# Autodesk Inventor assembly: Eto_Project
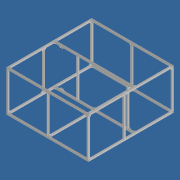
[picture p0: Inventor's stored thumbnail of the model, 180x180]
Saved by Autodesk Inventor 2020 (Build 240168000, 168)
## iProperties
Created: 2021-06-15
Part Number: Eto_Project
Description: CAx-IF Rec.Pracs.---Model Styling and Organization---1.2---2011-12-15
Document SubType Name: Assembly
Designer: ken113
Sending System: 3D_Kernel_IO2017 Sp2 by CT CoreTechnologie
Preprocessor: STEP Interface 2017 Sp2 by CT CoreTechnologie
Title: Eto_Project.stp
## Documents named in this file (68)
- D:\Document\Github\Eto_Project\Hardware\Asem\FRAMES\FramesEto_Project.iam
- D:\Document\Github\Eto_Project\Hardware\Asem\FRAMES\FramesHFS6-3030-1500.ipt
- D:\Document\Github\Eto_Project\Hardware\Asem\FRAMES\FramesHFS6-3030-690.ipt
- D:\Document\Github\Eto_Project\Hardware\Asem\FRAMES\FramesHBLFSN6-SET(1).iam
- D:\Document\Github\Eto_Project\Hardware\Asem\FRAMES\FramesHBLFSN6-SET(2).iam
- D:\Document\Github\Eto_Project\Hardware\Asem\FRAMES\FramesHBLFSN6-SET(3).iam
- D:\Document\Github\Eto_Project\Hardware\Asem\FRAMES\FramesHBLFSN6-SET(4).iam
- D:\Document\Github\Eto_Project\Hardware\Asem\FRAMES\FramesHBLFSN6-SET(5).iam
- D:\Document\Github\Eto_Project\Hardware\Asem\FRAMES\FramesHBLFSN6-SET(6).iam
- D:\Document\Github\Eto_Project\Hardware\Asem\FRAMES\FramesHBLFSN6-SET(7).iam
- D:\Document\Github\Eto_Project\Hardware\Asem\FRAMES\FramesHBLFSN6-SET(8).iam
- D:\Document\Github\Eto_Project\Hardware\Asem\FRAMES\FramesHBLFSN6-SET(9).iam
- D:\Document\Github\Eto_Project\Hardware\Asem\FRAMES\FramesHBLFSN6-SET(10).iam
- D:\Document\Github\Eto_Project\Hardware\Asem\FRAMES\FramesHBLFSN6-SET(11).iam
- D:\Document\Github\Eto_Project\Hardware\Asem\FRAMES\FramesHBLFSN6-SET(12).iam
- D:\Document\Github\Eto_Project\Hardware\Asem\FRAMES\FramesHBLFSN6-SET(13).iam
- D:\Document\Github\Eto_Project\Hardware\Asem\FRAMES\FramesHBLFSN6-SET(14).iam
- D:\Document\Github\Eto_Project\Hardware\Asem\FRAMES\FramesHBLFSN6-SET(15).iam
- D:\Document\Github\Eto_Project\Hardware\Asem\FRAMES\FramesHBLFSN6-SET(16).iam
- D:\Document\Github\Eto_Project\Hardware\Asem\FRAMES\FramesHBLFSN6-SET(17).iam
- D:\Document\Github\Eto_Project\Hardware\Asem\FRAMES\FramesHBLFSN6-SET(18).iam
- D:\Document\Github\Eto_Project\Hardware\Asem\FRAMES\FramesHBLFSN6-SET(19).iam
- D:\Document\Github\Eto_Project\Hardware\Asem\FRAMES\FramesHBLFSN6-SET(20).iam
- D:\Document\Github\Eto_Project\Hardware\Asem\FRAMES\FramesHBLFSN6-SET(21).iam
- D:\Document\Github\Eto_Project\Hardware\Asem\FRAMES\FramesHBLFSN6-SET(22).iam
- D:\Document\Github\Eto_Project\Hardware\Asem\FRAMES\FramesHBLFSN6-SET(23).iam
- D:\Document\Github\Eto_Project\Hardware\Asem\FRAMES\FramesHBLFSN6-SET(24).iam
- D:\Document\Github\Eto_Project\Hardware\Asem\FRAMES\FramesHFS6-3030-1440.ipt
- D:\Document\Github\Eto_Project\Hardware\Asem\FRAMES\FramesHBLFSN6-SET(25).iam
- D:\Document\Github\Eto_Project\Hardware\Asem\FRAMES\FramesHBLFSN6-SET(26).iam
- D:\Document\Github\Eto_Project\Hardware\Asem\FRAMES\FramesHBLFSN6-SET(27).iam
- D:\Document\Github\Eto_Project\Hardware\Asem\FRAMES\FramesHBLFSN6-SET(28).iam
- D:\Document\Github\Eto_Project\Hardware\Asem\FRAMES\FramesHBLFSN6-SET(29).iam
- D:\Document\Github\Eto_Project\Hardware\Asem\FRAMES\FramesHBLFSN6-SET(30).iam
- D:\Document\Github\Eto_Project\Hardware\Asem\FRAMES\FramesHBLFSN6-SET(31).iam
- D:\Document\Github\Eto_Project\Hardware\Asem\FRAMES\FramesHBLFSN6-SET(32).iam
- D:\Document\Github\Eto_Project\Hardware\Asem\FRAMES\FramesHBLFSN6-SET(33).iam
- D:\Document\Github\Eto_Project\Hardware\Asem\FRAMES\FramesHBLFSN6-SET(34).iam
- D:\Document\Github\Eto_Project\Hardware\Asem\FRAMES\FramesHBLFSN6-SET(35).iam
- D:\Document\Github\Eto_Project\Hardware\Asem\FRAMES\FramesHBLFSN6-SET(36).iam
- D:\Document\Github\Eto_Project\Hardware\Asem\FRAMES\FramesHFS6-3030-650.ipt
- D:\Document\Github\Eto_Project\Hardware\Asem\FRAMES\FramesHBLFSN6-SET(37).iam
- D:\Document\Github\Eto_Project\Hardware\Asem\FRAMES\FramesHBLFSN6-SET(38).iam
- D:\Document\Github\Eto_Project\Hardware\Asem\FRAMES\FramesHBLFSN6-SET(39).iam
- D:\Document\Github\Eto_Project\Hardware\Asem\FRAMES\FramesHBLFSN6-SET(40).iam
- D:\Document\Github\Eto_Project\Hardware\Asem\FRAMES\FramesHBLFSN6-SET(41).iam
- D:\Document\Github\Eto_Project\Hardware\Asem\FRAMES\FramesHBLFSN6-SET(42).iam
- D:\Document\Github\Eto_Project\Hardware\Asem\FRAMES\FramesHBLFSN6-SET(43).iam
- D:\Document\Github\Eto_Project\Hardware\Asem\FRAMES\FramesHBLFSN6-SET(44).iam
- D:\Document\Github\Eto_Project\Hardware\Asem\FRAMES\FramesHBLFSN6-SET(45).iam
- D:\Document\Github\Eto_Project\Hardware\Asem\FRAMES\FramesHFS6-3030-820.ipt
- D:\Document\Github\Eto_Project\Hardware\Asem\FRAMES\FramesHBLFSN6-SET(46).iam
- D:\Document\Github\Eto_Project\Hardware\Asem\FRAMES\FramesHBLFSN6-SET(47).iam
- D:\Document\Github\Eto_Project\Hardware\Asem\FRAMES\FramesHBLFSN6-SET(48).iam
- D:\Document\Github\Eto_Project\Hardware\Asem\FRAMES\FramesHBLFSN6-SET(49).iam
- D:\Document\Github\Eto_Project\Hardware\Asem\FRAMES\FramesHBLFSN6-SET(50).iam
- D:\Document\Github\Eto_Project\Hardware\Asem\FRAMES\FramesHBLFSN6-SET(51).iam
- D:\Document\Github\Eto_Project\Hardware\Asem\FRAMES\FramesHBLFSN6-SET(52).iam
- D:\Document\Github\Eto_Project\Hardware\Asem\FRAMES\FramesHBLFSN6-SET(53).iam
- D:\Document\Github\Eto_Project\Hardware\Asem\FRAMES\FramesHBLFSN6-SET(54).iam
- D:\Document\Github\Eto_Project\Hardware\Asem\FRAMES\FramesHBLFSN6-SET(55).iam
- D:\Document\Github\Eto_Project\Hardware\Asem\FRAMES\FramesHBLFSN6-SET(56).iam
- D:\Document\Github\Eto_Project\Hardware\Asem\FRAMES\FramesHBLFSN6-SET(57).iam
- D:\Document\Github\Eto_Project\Hardware\Asem\FRAMES\FramesHBLFSN6-SET(58).iam
- D:\Document\Github\Eto_Project\Hardware\Asem\FRAMES\FramesHBLFSN6-SET(59).iam
- D:\Document\Github\Eto_Project\Hardware\Asem\FRAMES\FramesHBLFSN6-SET(60).iam
- D:\Document\Github\Eto_Project\Hardware\Asem\FRAMES\FramesHBLFSN6-SET(61).iam
- D:\Document\Github\Eto_Project\Hardware\Asem\FRAMES\FramesHBLFSN6-SET(62).iam
## Components (84 placed, 67 different names)
1. HFS6-3030-1500
2. HFS6-3030-690
3. HBLFSN6-SET(1) [sub-assembly]
4. HFS6-3030-690:1
5. HBLFSN6-SET(2) [sub-assembly]
6. HFS6-3030-1500:1
7. HBLFSN6-SET(3) [sub-assembly]
8. HBLFSN6-SET(4) [sub-assembly]
9. HFS6-3030-1500:2 — フラッシュ:3, メイト:3, フラッシュ:4
10. HBLFSN6-SET(5) [sub-assembly]
11. HBLFSN6-SET(6) [sub-assembly]
12. HFS6-3030-1500:3
13. HBLFSN6-SET(7) [sub-assembly]
14. HBLFSN6-SET(8) [sub-assembly]
15. HFS6-3030-1500:4
16. HBLFSN6-SET(9) [sub-assembly]
17. HBLFSN6-SET(10) [sub-assembly]
18. HFS6-3030-1500:5 — フラッシュ:5, メイト:4
19. HBLFSN6-SET(11) [sub-assembly]
20. HBLFSN6-SET(12) [sub-assembly]
21. HFS6-3030-1500:6
22. HBLFSN6-SET(13) [sub-assembly]
23. HBLFSN6-SET(14) [sub-assembly]
24. HFS6-3030-1500:7
25. HBLFSN6-SET(15) [sub-assembly]
26. HBLFSN6-SET(16) [sub-assembly]
27. HFS6-3030-690:2
28. HBLFSN6-SET(17) [sub-assembly]
29. HBLFSN6-SET(18) [sub-assembly]
30. HBLFSN6-SET(19) [sub-assembly]
31. HBLFSN6-SET(20) [sub-assembly]
32. HFS6-3030-690:3
33. HBLFSN6-SET(21) [sub-assembly]
34. HBLFSN6-SET(22) [sub-assembly]
35. HBLFSN6-SET(23) [sub-assembly]
36. HBLFSN6-SET(24) [sub-assembly]
37. HFS6-3030-1440 — フラッシュ:1
38. HBLFSN6-SET(25) [sub-assembly]
39. HBLFSN6-SET(26) [sub-assembly]
40. HBLFSN6-SET(27) [sub-assembly]
41. HBLFSN6-SET(28) [sub-assembly]
42. HFS6-3030-690:4 — フラッシュ:5, メイト:4, フラッシュ:6
43. HBLFSN6-SET(29) [sub-assembly]
44. HBLFSN6-SET(30) [sub-assembly]
45. HBLFSN6-SET(31) [sub-assembly]
46. HBLFSN6-SET(32) [sub-assembly]
47. HFS6-3030-1440:1 — メイト:1, メイト:2, フラッシュ:2
48. HBLFSN6-SET(33) [sub-assembly]
49. HBLFSN6-SET(34) [sub-assembly]
50. HBLFSN6-SET(35) [sub-assembly]
51. HBLFSN6-SET(36) [sub-assembly]
52. HFS6-3030-650
53. HBLFSN6-SET(37) [sub-assembly]
54. HBLFSN6-SET(38) [sub-assembly]
55. HBLFSN6-SET(39) [sub-assembly]
56. HBLFSN6-SET(40) [sub-assembly]
57. HFS6-3030-690:5
58. HBLFSN6-SET(41) [sub-assembly]
59. HBLFSN6-SET(42) [sub-assembly]
60. HBLFSN6-SET(43) [sub-assembly]
61. HBLFSN6-SET(44) [sub-assembly]
62. HBLFSN6-SET(45) [sub-assembly]
63. HFS6-3030-820
64. HBLFSN6-SET(46) [sub-assembly]
65. HBLFSN6-SET(47) [sub-assembly]
66. HBLFSN6-SET(48) [sub-assembly]
67. HBLFSN6-SET(49) [sub-assembly]
68. HFS6-3030-690:6
69. HBLFSN6-SET(50) [sub-assembly]
70. HBLFSN6-SET(51) [sub-assembly]
71. HBLFSN6-SET(52) [sub-assembly]
72. HBLFSN6-SET(53) [sub-assembly]
73. HBLFSN6-SET(54) [sub-assembly]
74. HFS6-3030-690:8 — メイト:2, フラッシュ:2, フラッシュ:3
75. HBLFSN6-SET(59) [sub-assembly]
76. HBLFSN6-SET(60) [sub-assembly]
77. HBLFSN6-SET(61) [sub-assembly]
78. HBLFSN6-SET(62) [sub-assembly]
79. HFS6-3030-690:9 — メイト:3, フラッシュ:4, フラッシュ:6
80. HFS6-3030-690:7 — フラッシュ:1, メイト:1
81. HBLFSN6-SET(55) [sub-assembly]
82. HBLFSN6-SET(56) [sub-assembly]
83. HBLFSN6-SET(57) [sub-assembly]
84. HBLFSN6-SET(58) [sub-assembly]
## Relationships (10: Flush 6, Mate 4)
- フラッシュ:1 [Flush]: HFS6-3030-1440 ↔ HFS6-3030-690:7
- メイト:1 [Mate]: HFS6-3030-1440:1 ↔ HFS6-3030-690:7
- メイト:2 [Mate]: HFS6-3030-1440:1 ↔ HFS6-3030-690:8
- フラッシュ:2 [Flush]: HFS6-3030-1440:1 ↔ HFS6-3030-690:8
- フラッシュ:3 [Flush] (130 mm): HFS6-3030-1500:2 ↔ HFS6-3030-690:8
- メイト:3 [Mate]: HFS6-3030-1500:2 ↔ HFS6-3030-690:9
- フラッシュ:4 [Flush]: HFS6-3030-1500:2 ↔ HFS6-3030-690:9
- フラッシュ:5 [Flush]: HFS6-3030-1500:5 ↔ HFS6-3030-690:4
- メイト:4 [Mate]: HFS6-3030-1500:5 ↔ HFS6-3030-690:4
- フラッシュ:6 [Flush]: HFS6-3030-690:4 ↔ HFS6-3030-690:9
